# Autodesk Inventor assembly: 6in Wheel
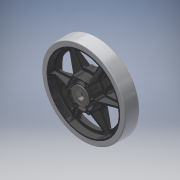
[picture p0: Inventor's stored thumbnail of the model, 180x180]
Saved by Autodesk Inventor 2018 (Build 220112000, 112)
## iProperties
Created: 2018-01-13
Part Number: 6in Wheel
Document SubType Name: Assembly
Designer: maste
Author: maste
## Documents named in this file (3)
- C:\Users\maste\Desktop\Drivebase 2018 Files 2\6in Wheel.iam
- C:\Users\maste\Desktop\Drivebase 2018 Files 2\2008-FIRST-Wheel.iam
- C:\Users\maste\Desktop\Drivebase 2018 Files 2\0_500_Hex_ID_x_1_125_OD_x_0_313_WD_Flanged_Bearing_v2_217-3875.ipt
## Components (2 placed, 2 different names)
1. 2008-FIRST-Wheel:1 [sub-assembly] — Mate:1, Mate:2, Rotation:1
2. 0_500_Hex_ID_x_1_125_OD_x_0_313_WD_Flanged_Bearing_v2_217-3875:1 — Mate:1, Mate:2, Rotation:1
## Relationships (3: Mate 2, RelateRotation 1)
- Mate:1: 2008-FIRST-Wheel:1 ↔ 0_500_Hex_ID_x_1_125_OD_x_0_313_WD_Flanged_Bearing_v2_217-3875:1
- Mate:2: 2008-FIRST-Wheel:1 ↔ 0_500_Hex_ID_x_1_125_OD_x_0_313_WD_Flanged_Bearing_v2_217-3875:1
- Rotation:1 [RelateRotation] (1 ul): 2008-FIRST-Wheel:1 ↔ 0_500_Hex_ID_x_1_125_OD_x_0_313_WD_Flanged_Bearing_v2_217-3875:1
